# Autodesk Inventor assembly: Base_Component_v2
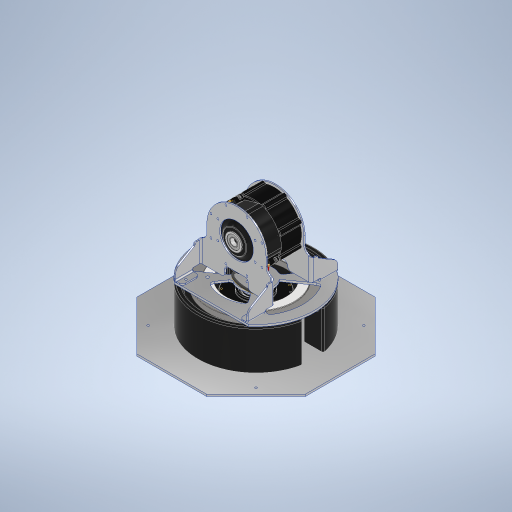
[picture p0: Inventor's stored thumbnail of the model, 512x512]
Saved by Autodesk Inventor 2024.3 (Build 283343010, 343A)
## iProperties
Created: 2025-09-25
Part Number: Base_Component_v2
Document SubType Name: Assembly
Designer: kshau
Author: kshau
## Documents named in this file (21)
- C:\Users\kshau\Documents\inventor\Create_ViperX\Create_ViperX_ALOHA\Base_Component_v2\Base_Component_v2.iam
- ArmBase_v2.iam
- C:\Users\kshau\Documents\inventor\Create_ViperX\Create_ViperX_ALOHA\Actuator\RS06\RS06\RS06.iam
- C:\Users\kshau\Documents\inventor\Create_ViperX\Create_ViperX_ALOHA\Base_Component_v2\basefixplate1_forR6.ipt
- C:\Users\kshau\Documents\inventor\Create_ViperX\Create_ViperX_ALOHA\Base_Component_v2\basefixplate2_forR6.ipt
- C:\Users\kshau\Documents\inventor\Create_ViperX\Create_ViperX_ALOHA\Base_Component_v2\basefixpart_forR6.ipt
- C:\Users\kshau\Documents\inventor\Create_ViperX\Create_ViperX_ALOHA\Base_Component_v2\servoplate_forR6.ipt
- C:\Users\kshau\Documents\inventor\Create_ViperX\Create_ViperX_ALOHA\Base_Component_v2\baseplate_R2toR6.ipt
- C:\Users\kshau\Documents\inventor\Create_ViperX\Create_ViperX_ALOHA\BasicParts\TurnTable\TurnTable_140\TurnTable_140.iam
- C:\Users\kshau\Documents\inventor\Create_ViperX\Create_ViperX_ALOHA\Base_Component\basespacer1.ipt
- C:\Users\kshau\Documents\inventor\Create_ViperX\Create_ViperX_ALOHA\Base_Component_v2\servoplate_forR2.ipt
- C:\Users\kshau\Documents\inventor\Create_ViperX\Create_ViperX_ALOHA\Actuator\RS02\RS02\RS02.iam
- C:\Users\kshau\Documents\inventor\Create_ViperX\Create_ViperX_ALOHA\NessesaryParts\ALSBF10-40-M4-N4\ALSBF10-40-M4-N4\ALSBF10-40-M4-N4.ipt
- C:\Users\kshau\Documents\inventor\Create_ViperX\Create_ViperX_ALOHA\Base_Component_v2\basepart2_forR2_v2.ipt
- C:\Users\kshau\Documents\inventor\Create_ViperX\Create_ViperX_ALOHA\Base_Component_v2\basespacer1.ipt
- C:\Users\kshau\Documents\inventor\Create_ViperX\Create_ViperX_ALOHA\Base_Component\basepart1_forR2.ipt
- C:\Users\kshau\Documents\inventor\Create_ViperX\Create_ViperX_ALOHA\BasicParts\Bearing\NMB_RF2210X2HH\RF-2210X2HH.iam
- C:\Users\kshau\Documents\inventor\Create_ViperX\Create_ViperX_ALOHA\Base_Component\Largebaseplate.ipt
- C:\Users\kshau\Documents\inventor\Create_ViperX\Create_ViperX_ALOHA\Base_Component_v2\baseparameter_v2.ipt
- C:\Users\kshau\Documents\inventor\Create_ViperX\Create_ViperX_ALOHA\Circuit\XT30(2+2)\XT30(2+2)\XT30(2+2).ipt
- C:\Users\kshau\Documents\inventor\Create_ViperX\Create_ViperX_ALOHA\Base_Component_v2\Base_Component_v2\AIP\ケーブル＆ハーネス\Base_Component_v2.Harness1.iam
## Components (29 placed, 18 different names)
1. RS06:1 [sub-assembly] — 回転:3, メイト:1, メイト:2, メイト:3, メイト:14, メイト:15, 回転:43, メイト:19, メイト:20, メイト:21, メイト:22, メイト:23
2. basefixplate1_forR6:1 — 回転:8, 回転:41, 回転:42, メイト:14, メイト:15, 回転:43
3. basefixplate2_forR6:1 — メイト:12, 回転:40
4. basefixpart_forR6:1 — 回転:3, メイト:1, メイト:11, 回転:40
5. servoplate_forR6:1 — メイト:2, メイト:3
6. baseplate_R2toR6:1 — 回転:8, 回転:15, 回転:16, 回転:28, メイト:4, 回転:41, フラッシュ:5, 回転:42, メイト:13
7. TurnTable_140:1 [sub-assembly] — 回転:9, 回転:10, 回転:30, 回転:31, 回転:32, 回転:33, メイト:6, メイト:8
8. basespacer1:1 — 回転:9, 回転:10, 回転:15, 回転:16
9. servoplate_forR2:1 — 回転:28, メイト:4, 回転:29, メイト:5
10. RS02:1 [sub-assembly] — 回転:29, メイト:5, メイト:7, メイト:9, 回転:37, 回転:38, メイト:16, メイト:17, メイト:18, メイト:24, メイト:25, メイト:26
11. ALSBF10-40-M4-N4:1 — 回転:30, 回転:35, フラッシュ:4
12. ALSBF10-40-M4-N4:2 — 回転:32, 回転:36, フラッシュ:2
13. ALSBF10-40-M4-N4:3 — 回転:33, リジッド:1, フラッシュ:3
14. ALSBF10-40-M4-N4:4 — 回転:31, 回転:34, フラッシュ:1
15. basepart2_forR2_v2:1 — メイト:6, メイト:7, メイト:10, メイト:13
16. basepart2_forR2_v2:2 — メイト:8, メイト:9, メイト:10
17. basespacer1:2 — 回転:34, フラッシュ:1
18. basespacer1:3 — 回転:35, フラッシュ:4
19. basespacer1:4 — リジッド:1, 回転:39, フラッシュ:3
20. basespacer1:5 — 回転:36, リジッド:2, フラッシュ:2
21. basepart1_forR2:1 — 回転:37, 回転:38
22. RF-2210X2HH:1 [sub-assembly] — メイト:11, メイト:12
23. Largebaseplate:1 — 回転:39, リジッド:2, フラッシュ:5
24. baseparameter_v2:1
25. XT30(2+2):1 — メイト:16, メイト:17, メイト:18
26. XT30(2+2):2 — メイト:19, メイト:20, メイト:21, フラッシュ:6
27. XT30(2+2):3 — メイト:22, メイト:23, フラッシュ:6
28. XT30(2+2):4 — メイト:24, メイト:25, メイト:26
29. Harness1 [sub-assembly]
## Relationships (56: Mate 26, RevoluteJoint 22, Flush 6, WeldJoint 2)
- 回転:3 [RevoluteJoint]: RS06:1 ↔ basefixpart_forR6:1
- メイト:1 [Mate]: RS06:1 ↔ basefixpart_forR6:1
- メイト:2 [Mate]: RS06:1 ↔ servoplate_forR6:1
- メイト:3 [Mate]: RS06:1 ↔ servoplate_forR6:1
- 回転:8 [RevoluteJoint]: basefixplate1_forR6:1 ↔ baseplate_R2toR6:1
- 回転:9 [RevoluteJoint]: TurnTable_140:1 ↔ basespacer1:1
- 回転:10 [RevoluteJoint]: TurnTable_140:1 ↔ basespacer1:1
- 回転:15 [RevoluteJoint]: baseplate_R2toR6:1 ↔ basespacer1:1
- 回転:16 [RevoluteJoint]: baseplate_R2toR6:1 ↔ basespacer1:1
- 回転:28 [RevoluteJoint]: baseplate_R2toR6:1 ↔ servoplate_forR2:1
- メイト:4 [Mate]: baseplate_R2toR6:1 ↔ servoplate_forR2:1
- 回転:29 [RevoluteJoint]: servoplate_forR2:1 ↔ RS02:1
- メイト:5 [Mate]: servoplate_forR2:1 ↔ RS02:1
- 回転:30 [RevoluteJoint]: TurnTable_140:1 ↔ ALSBF10-40-M4-N4:1
- 回転:31 [RevoluteJoint]: TurnTable_140:1 ↔ ALSBF10-40-M4-N4:4
- 回転:32 [RevoluteJoint]: TurnTable_140:1 ↔ ALSBF10-40-M4-N4:2
- 回転:33 [RevoluteJoint]: TurnTable_140:1 ↔ ALSBF10-40-M4-N4:3
- メイト:6 [Mate]: TurnTable_140:1 ↔ basepart2_forR2_v2:1
- メイト:7 [Mate]: RS02:1 ↔ basepart2_forR2_v2:1
- メイト:8 [Mate]: TurnTable_140:1 ↔ basepart2_forR2_v2:2
- メイト:9 [Mate]: RS02:1 ↔ basepart2_forR2_v2:2
- メイト:10 [Mate] (30 mm): basepart2_forR2_v2:1 ↔ basepart2_forR2_v2:2
- 回転:34 [RevoluteJoint]: ALSBF10-40-M4-N4:4 ↔ basespacer1:2
- リジッド:1 [WeldJoint]: ALSBF10-40-M4-N4:3 ↔ basespacer1:4
- 回転:35 [RevoluteJoint]: ALSBF10-40-M4-N4:1 ↔ basespacer1:3
- 回転:36 [RevoluteJoint]: ALSBF10-40-M4-N4:2 ↔ basespacer1:5
- 回転:37 [RevoluteJoint]: RS02:1 ↔ basepart1_forR2:1
- 回転:38 [RevoluteJoint]: RS02:1 ↔ basepart1_forR2:1
- メイト:11 [Mate]: basefixpart_forR6:1 ↔ RF-2210X2HH:1
- メイト:12 [Mate]: basefixplate2_forR6:1 ↔ RF-2210X2HH:1
- 回転:39 [RevoluteJoint]: basespacer1:4 ↔ Largebaseplate:1
- リジッド:2 [WeldJoint]: basespacer1:5 ↔ Largebaseplate:1
- 回転:40 [RevoluteJoint]: basefixplate2_forR6:1 ↔ basefixpart_forR6:1
- 回転:41 [RevoluteJoint]: basefixplate1_forR6:1 ↔ baseplate_R2toR6:1
- フラッシュ:1 [Flush]: ALSBF10-40-M4-N4:4 ↔ basespacer1:2
- フラッシュ:2 [Flush]: ALSBF10-40-M4-N4:2 ↔ basespacer1:5
- フラッシュ:3 [Flush]: ALSBF10-40-M4-N4:3 ↔ basespacer1:4
- フラッシュ:4 [Flush]: ALSBF10-40-M4-N4:1 ↔ basespacer1:3
- フラッシュ:5 [Flush] (-58.5 mm): baseplate_R2toR6:1 ↔ Largebaseplate:1
- 回転:42 [RevoluteJoint]: basefixplate1_forR6:1 ↔ baseplate_R2toR6:1
- メイト:13 [Mate] (-51.5 mm): baseplate_R2toR6:1 ↔ basepart2_forR2_v2:1
- メイト:14 [Mate]: RS06:1 ↔ basefixplate1_forR6:1
- メイト:15 [Mate]: RS06:1 ↔ basefixplate1_forR6:1
- 回転:43 [RevoluteJoint]: RS06:1 ↔ basefixplate1_forR6:1
- メイト:16 [Mate]: RS02:1 ↔ XT30(2+2):1
- メイト:17 [Mate] (0.1 mm): RS02:1 ↔ XT30(2+2):1
- メイト:18 [Mate] (0.3 mm): RS02:1 ↔ XT30(2+2):1
- メイト:19 [Mate]: RS06:1 ↔ XT30(2+2):2
- メイト:20 [Mate] (1 mm): RS06:1 ↔ XT30(2+2):2
- メイト:21 [Mate] (1.35 mm): RS06:1 ↔ XT30(2+2):2
- メイト:22 [Mate]: RS06:1 ↔ XT30(2+2):3
- メイト:23 [Mate] (1 mm): RS06:1 ↔ XT30(2+2):3
- フラッシュ:6 [Flush]: XT30(2+2):2 ↔ XT30(2+2):3
- メイト:24 [Mate]: RS02:1 ↔ XT30(2+2):4
- メイト:25 [Mate] (0.13 mm): RS02:1 ↔ XT30(2+2):4
- メイト:26 [Mate]: RS02:1 ↔ XT30(2+2):4
